# Autodesk Inventor assembly: tandwiel_MIROR1
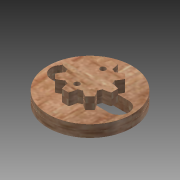
[picture p0: Inventor's stored thumbnail of the model, 180x180]
Saved by Autodesk Inventor 2015 (Build 190159000, 159)
## iProperties
Created: 2016-01-31
Part Number: tandwiel_MIROR1
Document SubType Name: Assembly
Designer: david
Author: david
## Documents named in this file (3)
- Z:\gip\Inventor\generatie 7\motor v2\tandwiel\tandwiel_MIROR1.iam
- Z:\gip\Inventor\generatie 7\motor v2\tandwiel\1_MIROR1.ipt
- Z:\gip\Inventor\generatie 7\motor v2\tandwiel\tandwiel(ja)_MIROR1.ipt
## Components (4 placed, 2 different names)
1. 1_MIROR1:1 — Flush:1, Mate:2, Mate:1
2. 1_MIROR1:2 — Flush:1, Mate:2, Mate:1, Flush:2, Mate:6, Mate:5
3. tandwiel(ja)_MIROR1:1 — Flush:2, Mate:4, Mate:3
4. tandwiel(ja)_MIROR1:2 — Mate:6, Mate:5, Mate:4, Mate:3
## Relationships (8: Mate 7, Flush 1)
- Flush:1: 1_MIROR1:1 ↔ 1_MIROR1:2
- Mate:2: 1_MIROR1:1 ↔ 1_MIROR1:2
- Mate:1: 1_MIROR1:1 ↔ 1_MIROR1:2
- Flush:2 [Mate]: 1_MIROR1:2 ↔ tandwiel(ja)_MIROR1:1
- Mate:6: 1_MIROR1:2 ↔ tandwiel(ja)_MIROR1:2
- Mate:5: 1_MIROR1:2 ↔ tandwiel(ja)_MIROR1:2
- Mate:4: tandwiel(ja)_MIROR1:1 ↔ tandwiel(ja)_MIROR1:2
- Mate:3: tandwiel(ja)_MIROR1:1 ↔ tandwiel(ja)_MIROR1:2
